# Autodesk Inventor assembly: MolexFixClip_Assy
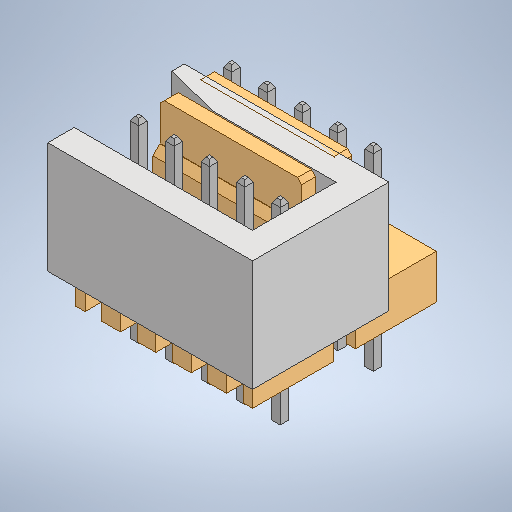
[picture p0: Inventor's stored thumbnail of the model, 512x512]
Saved by Autodesk Inventor 2025.1 (Build 291241000, 241)
## iProperties
Created: 2026-05-09
Part Number: MolexFixClip_Assy
Document SubType Name: Assembly
Designer: User
Author: User
## Documents named in this file (4)
- D:\One Drive\OneDrive - Politeknik Sultan Salahuddin Abdul Aziz Shah\Documents\Inventor\RobosotPSA\MolexFixClip_Assy.iam
- D:\One Drive\OneDrive - Politeknik Sultan Salahuddin Abdul Aziz Shah\Documents\Inventor\RobosotPSA\Molex-2.54-5pin\Molex-2.54-5pin\Molex-2.54-5pin.ipt
- D:\One Drive\OneDrive - Politeknik Sultan Salahuddin Abdul Aziz Shah\Documents\Inventor\RobosotPSA\MolexClipper.ipt
- D:\One Drive\OneDrive - Politeknik Sultan Salahuddin Abdul Aziz Shah\Documents\Inventor\RobosotPSA\MolexClipper_vertical.ipt
## Components (4 placed, 3 different names)
1. Molex-2.54-5pin:1 — Flush:1, Flush:2, Flush:3, Flush:4, Mate:1
2. MolexClipper:1 — Flush:1
3. MolexClipper_vertical:1 — Flush:2
4. Molex-2.54-5pin:2 — Flush:3, Flush:4, Mate:1
## Relationships (5: Flush 4, Mate 1)
- Flush:1: Molex-2.54-5pin:1 ↔ MolexClipper:1
- Flush:2: Molex-2.54-5pin:1 ↔ MolexClipper_vertical:1
- Flush:3: Molex-2.54-5pin:1 ↔ Molex-2.54-5pin:2
- Flush:4: Molex-2.54-5pin:1 ↔ Molex-2.54-5pin:2
- Mate:1 (1.6 mm): Molex-2.54-5pin:1 ↔ Molex-2.54-5pin:2
